# Autodesk Inventor assembly: Tracker Wheel
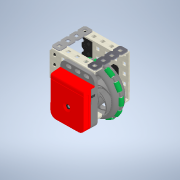
[picture p0: Inventor's stored thumbnail of the model, 180x180]
Saved by Autodesk Inventor 2020 (Build 240168000, 168)
## iProperties
Created: 2019-09-01
Part Number: Tracker Wheel
Document SubType Name: Assembly
Designer: Corey
Author: Corey
## Documents named in this file (7)
- C:\Users\Corey\Google Drive\2019_2020 Tower Takeover\CAD\Tracker Wheel.iam
- C:\Users\Corey\Google Drive\2019_2020 Tower Takeover\CAD\Parts\Motion\Wheels & Rollers\2.75'' Omni-Directional Wheel.iam
- C:\Users\Corey\Google Drive\2019_2020 Tower Takeover\CAD\Parts\Electronics\Optical Shaft Encoder.iam
- C:\Users\Corey\Google Drive\2019_2020 Tower Takeover\CAD\Parts\Structure\1 Wide Bar\Bar 1x4.ipt
- C:\Users\Corey\Google Drive\2019_2020 Tower Takeover\CAD\Parts\Motion\Bearing Flat.ipt
- C:\Users\Corey\Google Drive\2019_2020 Tower Takeover\CAD\Parts\Motion\Drive Shafts\Drive Shaft 3''.ipt
- C:\Users\Corey\Google Drive\2019_2020 Tower Takeover\CAD\Parts\Structure\C-Channels\Aluminum\5-Wide\Aluminum C-Channel 1x5x1x5.ipt
## Components (10 placed, 6 different names)
1. 2.75'' Omni-Directional Wheel:1 [sub-assembly] — Mate:10, Mate:11, Flush:7
2. Bearing Flat:1 — Insert:1, Insert:2, Insert:3
3. Drive Shaft 3'':1 — Mate:10, Mate:11, Flush:7, Insert:3
4. Optical Shaft Encoder:1 [sub-assembly] — Mate:22, Flush:27, Mate:23
5. Aluminum C-Channel 1x5x1x5:1 — Mate:20, Mate:21, Flush:25, Flush:26, Mate:22, Flush:27, Mate:23, Insert:6, Insert:7
6. Aluminum C-Channel 1x5x1x5:2 — Flush:21, Flush:22, Mate:19, Flush:23, Flush:24, Insert:1, Insert:2, Insert:4, Insert:5
7. Bearing Flat:5 — Insert:4, Insert:5
8. Bearing Flat:6 — Insert:6, Insert:7
9. Bar 1x4:5 — Flush:21, Flush:22, Mate:20
10. Bar 1x4:6 — Mate:19, Flush:23, Flush:24, Mate:21, Flush:25, Flush:26
## Relationships (22: Flush 8, Mate 7, Insert 7)
- Mate:10: 2.75'' Omni-Directional Wheel:1 ↔ Drive Shaft 3'':1
- Mate:11: 2.75'' Omni-Directional Wheel:1 ↔ Drive Shaft 3'':1
- Flush:7 (22.098 mm): 2.75'' Omni-Directional Wheel:1 ↔ Drive Shaft 3'':1
- Flush:21: Aluminum C-Channel 1x5x1x5:2 ↔ Bar 1x4:5
- Flush:22: Aluminum C-Channel 1x5x1x5:2 ↔ Bar 1x4:5
- Mate:19: Aluminum C-Channel 1x5x1x5:2 ↔ Bar 1x4:6
- Flush:23: Aluminum C-Channel 1x5x1x5:2 ↔ Bar 1x4:6
- Flush:24: Aluminum C-Channel 1x5x1x5:2 ↔ Bar 1x4:6
- Mate:20: Aluminum C-Channel 1x5x1x5:1 ↔ Bar 1x4:5
- Mate:21: Aluminum C-Channel 1x5x1x5:1 ↔ Bar 1x4:6
- Flush:25: Aluminum C-Channel 1x5x1x5:1 ↔ Bar 1x4:6
- Flush:26: Aluminum C-Channel 1x5x1x5:1 ↔ Bar 1x4:6
- Mate:22: Optical Shaft Encoder:1 ↔ Aluminum C-Channel 1x5x1x5:1
- Flush:27: Optical Shaft Encoder:1 ↔ Aluminum C-Channel 1x5x1x5:1
- Mate:23 (1.016 mm): Optical Shaft Encoder:1 ↔ Aluminum C-Channel 1x5x1x5:1
- Insert:1: Bearing Flat:1 ↔ Aluminum C-Channel 1x5x1x5:2
- Insert:2: Bearing Flat:1 ↔ Aluminum C-Channel 1x5x1x5:2
- Insert:3 (-6.35 mm): Bearing Flat:1 ↔ Drive Shaft 3'':1
- Insert:4: Aluminum C-Channel 1x5x1x5:2 ↔ Bearing Flat:5
- Insert:5: Aluminum C-Channel 1x5x1x5:2 ↔ Bearing Flat:5
- Insert:6: Aluminum C-Channel 1x5x1x5:1 ↔ Bearing Flat:6
- Insert:7: Aluminum C-Channel 1x5x1x5:1 ↔ Bearing Flat:6
